# Autodesk Inventor assembly: Front Crossbrace
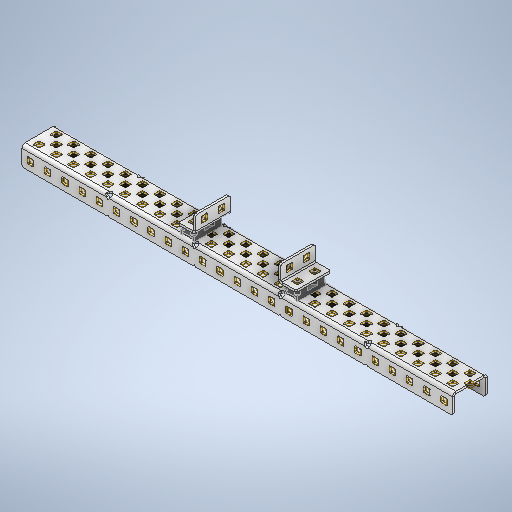
[picture p0: Inventor's stored thumbnail of the model, 512x512]
Saved by Autodesk Inventor 2025.2 (Build 292293000, 293)
## iProperties
Created: 2025-04-02
Part Number: Front Crossbrace
Document SubType Name: Assembly
Designer: avere
Author: avere
## Documents named in this file (4)
- D:\vex\cad\v5\Drivetrain\Braces\Front Crossbrace.iam
- D:\vex\cad\VEX-CAD-Inventor\Structure\C Channel\Aluminum 1x2x1\Alu C 1x2x1x25.ipt
- D:\vex\cad\VEX-CAD-Inventor\Structure\Angle\Aluminum 1x1\Alu Angle 1x1x2.ipt
- D:\vex\cad\VEX-CAD-Inventor\Motion\Shaft LS\Bearing Flat - Cut.ipt
## Components (5 placed, 3 different names)
1. Alu C 1x2x1x25:1 — Mate:1, Mate:2, Mate:3, Insert:1, Mate:4, Insert:2, Mate:5, Insert:3, Insert:4
2. Alu Angle 1x1x2:1 — Insert:1, Mate:4, Mate:6
3. Alu Angle 1x1x2:2 — Insert:2, Mate:5, Mate:7
4. Bearing Flat - Cut:1 — Insert:3, Mate:6
5. Bearing Flat - Cut:2 — Insert:4, Mate:7
## Relationships (11: Mate 7, Insert 4)
- Mate:1 (25.4 mm): Alu C 1x2x1x25:1
- Mate:2 (-158.75 mm): Alu C 1x2x1x25:1
- Mate:3 (50.8 mm): Alu C 1x2x1x25:1
- Insert:1 (6.35 mm): Alu C 1x2x1x25:1 ↔ Alu Angle 1x1x2:1
- Mate:4: Alu C 1x2x1x25:1 ↔ Alu Angle 1x1x2:1
- Insert:2 (6.35 mm): Alu C 1x2x1x25:1 ↔ Alu Angle 1x1x2:2
- Mate:5: Alu C 1x2x1x25:1 ↔ Alu Angle 1x1x2:2
- Insert:3: Alu C 1x2x1x25:1 ↔ Bearing Flat - Cut:1
- Mate:6: Alu Angle 1x1x2:1 ↔ Bearing Flat - Cut:1
- Insert:4: Alu C 1x2x1x25:1 ↔ Bearing Flat - Cut:2
- Mate:7: Alu Angle 1x1x2:2 ↔ Bearing Flat - Cut:2
